# Autodesk Inventor assembly: Assembly1
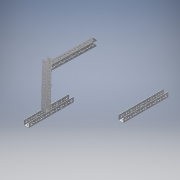
[picture p0: Inventor's stored thumbnail of the model, 180x180]
Saved by Autodesk Inventor 2016 (Build 200138000, 138)
## iProperties
Created: 2017-03-14
Part Number: Assembly1
Document SubType Name: Assembly
Designer: 293746
Author: 293746
## Documents named in this file (2)
- \\stushare\home\293746\Documents\Assembly1.iam
- C:\Users\293746\Desktop\FTC CAD Library\Channel\288mm Channel.ipt
## Components (4 placed, 1 different names)
1. 288mm Channel:1 — Mate:1, Mate:2, Mate:3, Mate:4
2. 288mm Channel:2 — Mate:1, Mate:2, Mate:3, Mate:4
3. 288mm Channel:3
4. 288mm Channel:4
## Relationships (4: Mate 4)
- Mate:1: 288mm Channel:1 ↔ 288mm Channel:2
- Mate:2: 288mm Channel:1 ↔ 288mm Channel:2
- Mate:3: 288mm Channel:1 ↔ 288mm Channel:2
- Mate:4: 288mm Channel:1 ↔ 288mm Channel:2
